# Autodesk Inventor assembly: feed-bpsupassy
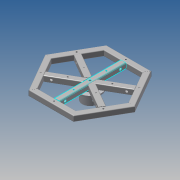
[picture p0: Inventor's stored thumbnail of the model, 180x180]
Saved by Autodesk Inventor 2013 SP2 (Build 170200200, 200)
## iProperties
Company: HERA Project
Created: 2013-06-27
Part Number: feed-bpsupassy
Document SubType Name: Assembly
Designer: David DeBoer
Description: Feed backplane support assembly
Author: David DeBoer
Title: Feed backplane support
## Documents named in this file (6)
- C:\Users\Dave\Desktop\hera-cad\feed\feed-bpsupassy.iam
- C:\Users\Dave\Desktop\hera-cad\feed\feed-bpsupxp.ipt
- C:\Users\Dave\Desktop\hera-cad\feed\feed-bpsuppc.ipt
- C:\Users\Dave\Desktop\hera-cad\feed\feed-bpsupip.ipt
- C:\Users\Dave\Desktop\hera-cad\feed\feed-bpsupip2.ipt
- C:\Users\Dave\Desktop\hera-cad\feed\collar.ipt
## Components (12 placed, 5 different names)
1. feed-bpsupxp:1 — Mate:1, Mate:3, Mate:4, Insert:1
2. collar:1 — Insert:1
3. feed-bpsuppc:1 — Mate:1
4. feed-bpsuppc:2
5. feed-bpsuppc:3
6. feed-bpsuppc:4
7. feed-bpsuppc:5
8. feed-bpsuppc:6
9. feed-bpsupip:2 — Mate:3
10. feed-bpsupip:3
11. feed-bpsupip2:1 — Mate:4
12. feed-bpsupip2:2
## Component patterns: outer (6 elements), inner1 (2 elements), inner2 (2 elements)
## Relationships (4: Mate 3, Insert 1)
- Mate:1: feed-bpsupxp:1 ↔ feed-bpsuppc:1
- Mate:3: feed-bpsupxp:1 ↔ feed-bpsupip:2
- Mate:4: feed-bpsupxp:1 ↔ feed-bpsupip2:1
- Insert:1: feed-bpsupxp:1 ↔ collar:1
